# Autodesk Inventor assembly: コリメート用レンズ_蛍光
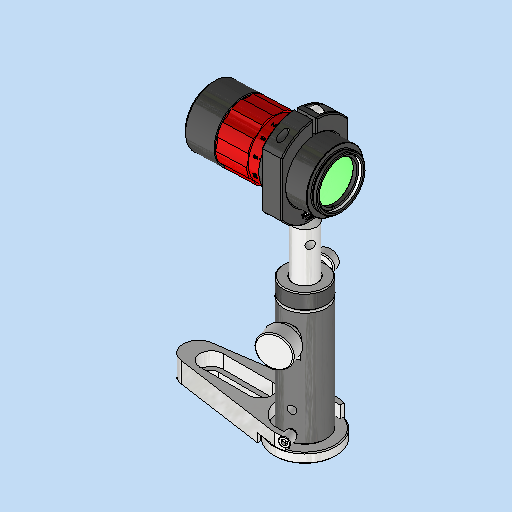
[picture p0: Inventor's stored thumbnail of the model, 512x512]
Saved by Autodesk Inventor 2025 (Build 290162000, 162)
## iProperties
Created: 2023-01-12
Part Number: コリメート用レンズ_蛍光
Document SubType Name: Assembly
Designer: Hiroma Goda
Author: Hiroma Goda
## Documents named in this file (7)
- C:\Users\queez\Dropbox\Drawings\PIHTI\ContentCenter\Optics\collimator.iam
- C:\Users\queez\Dropbox\Drawings\PIHTI\ContentCenter\Optics\PSCS-11.5UU.ipt
- C:\Users\queez\Dropbox\Drawings\PIHTI\ContentCenter\Optics\PSA-M16.ipt
- C:\Users\queez\Dropbox\Drawings\PIHTI\ContentCenter\Optics\BRS-12-60.ipt
- C:\Users\queez\Dropbox\Drawings\PIHTI\ContentCenter\Optics\ROC-12-60.ipt
- C:\Users\queez\Dropbox\Drawings\PIHTI\ContentCenter\Optics\C40FC-A-Step.ipt
- C:\Users\queez\Dropbox\Drawings\PIHTI\ContentCenter\Optics\SM1RC_M-Step.ipt
## Components (6 placed, 6 different names)
1. PSCS-11.5UU:1 — メイト:5, メイト:6
2. PSA-M16:1 — メイト:3, メイト:4, メイト:5
3. BRS-12-60:1 — メイト:3, メイト:4, メイト:6, メイト:10, メイト:14
4. ROC-12-60:1 — メイト:10, メイト:11, メイト:12
5. C40FC-A-Step:1 — メイト:13, フラッシュ:1
6. SM1RC_M-Step:1 — メイト:11, メイト:12, メイト:13, フラッシュ:1, メイト:14
## Relationships (10: Mate 9, Flush 1)
- メイト:3 [Mate]: PSA-M16:1 ↔ BRS-12-60:1
- メイト:4 [Mate]: PSA-M16:1 ↔ BRS-12-60:1
- メイト:5 [Mate]: PSCS-11.5UU:1 ↔ PSA-M16:1
- メイト:6 [Mate]: PSCS-11.5UU:1 ↔ BRS-12-60:1
- メイト:10 [Mate]: BRS-12-60:1 ↔ ROC-12-60:1
- メイト:11 [Mate]: ROC-12-60:1 ↔ SM1RC_M-Step:1
- メイト:12 [Mate]: ROC-12-60:1 ↔ SM1RC_M-Step:1
- メイト:13 [Mate]: C40FC-A-Step:1 ↔ SM1RC_M-Step:1
- フラッシュ:1 [Flush] (-10 mm): C40FC-A-Step:1 ↔ SM1RC_M-Step:1
- メイト:14 [Mate] (27.9 mm): BRS-12-60:1 ↔ SM1RC_M-Step:1
